# Autodesk Inventor assembly: Space
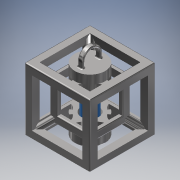
[picture p0: Inventor's stored thumbnail of the model, 180x180]
Saved by Autodesk Inventor 2019 (Build 230136000, 136)
## iProperties
Created: 2019-05-02
Part Number: Space
Document SubType Name: Assembly
Designer: Jorian Brusind
Author: Jorian Brusind
## Documents named in this file (3)
- C:\Users\Jorian Brusind\Documents\GitHub\PersonalProjects\Inventor Projects\Infinity\Space.iam
- C:\Users\Jorian Brusind\Documents\GitHub\PersonalProjects\Inventor Projects\Infinity\Inner.ipt
- C:\Users\Jorian Brusind\Documents\GitHub\PersonalProjects\Inventor Projects\Infinity\Blue.ipt
## Components (2 placed, 2 different names)
1. Inner:1 — Mate:1, Mate:2
2. Blue:1 — Mate:1, Mate:2
## Relationships (2: Mate 2)
- Mate:1: Inner:1 ↔ Blue:1
- Mate:2: Inner:1 ↔ Blue:1
